# Autodesk Inventor assembly: 方向変換用ミラー
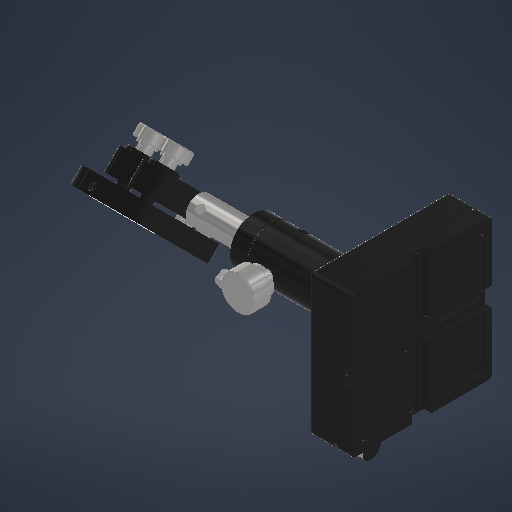
[picture p0: Inventor's stored thumbnail of the model, 512x512]
Saved by Autodesk Inventor 2026 (Build 300175050, 175E)
## iProperties
Created: 2025-07-11
Part Number: 方向変換用ミラー
Document SubType Name: Assembly
Designer: jin20
Author: jin20
## Documents named in this file (4)
- C:\Users\jin20\Documents\装置CAD\RamanSystem\方向変換用ミラー.iam
- C:\Users\jin20\Documents\装置CAD\RamanSystem\Optics\ミラー.iam
- C:\Users\jin20\Documents\装置CAD\RamanSystem\Optics\ロッドスタンド.ipt
- C:\Users\jin20\Documents\装置CAD\RamanSystem\Stage\マグネットベース.ipt
## Components (3 placed, 3 different names)
1. ミラー:1 [sub-assembly] — 回転:1
2. ロッドスタンド:1 — 挿入:1, 回転:1
3. マグネットベース:1 — 挿入:1
## Relationships (2: Insert 1, RevoluteJoint 1)
- 挿入:1 [Insert]: ロッドスタンド:1 ↔ マグネットベース:1
- 回転:1 [RevoluteJoint] (25 mm): ミラー:1 ↔ ロッドスタンド:1
